# Autodesk Inventor assembly: 2101_Tx_Coil_Spacer_Assm_V1
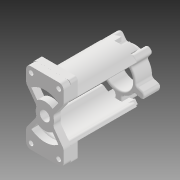
[picture p0: Inventor's stored thumbnail of the model, 180x180]
Saved by Autodesk Inventor 2021 (Build 250183000, 183)
## iProperties
Created: 2022-08-11
Part Number: 2101_Tx_Coil_Spacer_Assm_V1
Document SubType Name: Assembly
Designer: Eli
Author: Eli
## Documents named in this file (4)
- C:\Users\Eli\Documents\GitHub\MPS\Inventor Parts\MPSV2\2xxx Coil Formers and Parts\21xx Tx Coil\210x Tx Coil Solenoid Former\2101_Tx_Coil_Spacer_Assm_V1.iam
- C:\Users\Eli\Documents\GitHub\MPS\Inventor Parts\MPSV2\2xxx Coil Formers and Parts\21xx Tx Coil\210x Tx Coil Solenoid Former\2102_Tx_Coil_Fins_V1.ipt
- C:\Users\Eli\Documents\GitHub\MPS\Inventor Parts\MPSV2\2xxx Coil Formers and Parts\21xx Tx Coil\210x Tx Coil Solenoid Former\2103_Tx_CoilFin_Spacer_V1.ipt
- C:\Users\Eli\Documents\GitHub\MPS\Inventor Parts\MPSV2\2xxx Coil Formers and Parts\21xx Tx Coil\210x Tx Coil Solenoid Former\2104_Tx_CoilBackPlate_V1.ipt
## Components (4 placed, 3 different names)
1. 2102_Tx_Coil_Fins_V1:1 — Mate:2, Mate:3, Mate:4, Mate:6, Mate:7, Mate:8, Angle:1
2. 2103_Tx_CoilFin_Spacer_V1:1 — Mate:5, Flush:1, Flush:2, Mate:7, Flush:3, Flush:4
3. 2103_Tx_CoilFin_Spacer_V1:2 — Flush:1, Mate:6, Flush:2, Mate:8, Angle:1, Flush:3
4. 2104_Tx_CoilBackPlate_V1:1 — Flush:4
## Relationships (12: Mate 7, Flush 4, Angle 1)
- Mate:2: 2102_Tx_Coil_Fins_V1:1
- Mate:3: 2102_Tx_Coil_Fins_V1:1
- Mate:4: 2102_Tx_Coil_Fins_V1:1
- Mate:5: 2103_Tx_CoilFin_Spacer_V1:1
- Flush:1: 2103_Tx_CoilFin_Spacer_V1:1 ↔ 2103_Tx_CoilFin_Spacer_V1:2
- Mate:6: 2102_Tx_Coil_Fins_V1:1 ↔ 2103_Tx_CoilFin_Spacer_V1:2
- Flush:2: 2103_Tx_CoilFin_Spacer_V1:1 ↔ 2103_Tx_CoilFin_Spacer_V1:2
- Mate:7: 2102_Tx_Coil_Fins_V1:1 ↔ 2103_Tx_CoilFin_Spacer_V1:1
- Mate:8: 2102_Tx_Coil_Fins_V1:1 ↔ 2103_Tx_CoilFin_Spacer_V1:2
- Angle:1 (180 deg): 2102_Tx_Coil_Fins_V1:1 ↔ 2103_Tx_CoilFin_Spacer_V1:2
- Flush:3: 2103_Tx_CoilFin_Spacer_V1:1 ↔ 2103_Tx_CoilFin_Spacer_V1:2
- Flush:4: 2103_Tx_CoilFin_Spacer_V1:1 ↔ 2104_Tx_CoilBackPlate_V1:1
